# Autodesk Inventor assembly: leg_1
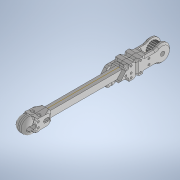
[picture p0: Inventor's stored thumbnail of the model, 180x180]
Saved by Autodesk Inventor 2020 (Build 240168000, 168)
## iProperties
Created: 2019-05-01
Part Number: leg_1
Document SubType Name: Assembly
Designer: psrob
Author: psrob
## Documents named in this file (8)
- E:\projects-2\project dog gen2\hardware\leg_bone_1.iam
- E:\projects-2\project dog gen2\hardware\leg_down_2.ipt
- E:\projects-2\project dog gen2\hardware\carbon_fiber_6.ipt
- E:\projects-2\project dog gen2\hardware\leg_down_3.ipt
- E:\projects-2\project dog gen2\hardware\leg_hip_1.ipt
- E:\projects-2\project dog gen2\hardware\leg_down_s1.ipt
- E:\projects-2\project dog gen2\hardware\leg_down_s1_MIR.ipt
- E:\projects-2\project dog gen2\hardware\leg_down_s3_l.ipt
## Components (8 placed, 7 different names)
1. carbon_fiber_6:1 — Mate:1, Mate:2, Mate:3, Flush:1, Mate:4, Mate:5, Flush:2, Mate:6, Mate:8, Mate:9
2. leg_down_2:1 — Mate:1, Mate:2, Mate:3, Insert:1, Insert:2, Mate:10
3. leg_down_3:1 — Insert:1, Insert:2, Mate:7
4. leg_hip_1:1 — Flush:1, Mate:4, Mate:5, Insert:3, Insert:4
5. leg_hip_1:2 — Insert:3, Insert:4
6. leg_down_s1:1 — Flush:2, Mate:6, Mate:7, Mate:11, Insert:5, Insert:6
7. leg_down_s1_MIR:1 — Mate:8, Mate:9, Mate:10
8. leg_down_s3_l:1 — Mate:11, Insert:5, Insert:6
## Relationships (19: Mate 11, Insert 6, Flush 2)
- Mate:1: carbon_fiber_6:1 ↔ leg_down_2:1
- Mate:2: carbon_fiber_6:1 ↔ leg_down_2:1
- Mate:3: carbon_fiber_6:1 ↔ leg_down_2:1
- Insert:1: leg_down_2:1 ↔ leg_down_3:1
- Insert:2: leg_down_2:1 ↔ leg_down_3:1
- Flush:1: carbon_fiber_6:1 ↔ leg_hip_1:1
- Mate:4: carbon_fiber_6:1 ↔ leg_hip_1:1
- Mate:5: carbon_fiber_6:1 ↔ leg_hip_1:1
- Insert:3: leg_hip_1:1 ↔ leg_hip_1:2
- Insert:4: leg_hip_1:1 ↔ leg_hip_1:2
- Flush:2: carbon_fiber_6:1 ↔ leg_down_s1:1
- Mate:6: carbon_fiber_6:1 ↔ leg_down_s1:1
- Mate:7: leg_down_3:1 ↔ leg_down_s1:1
- Mate:8: carbon_fiber_6:1 ↔ leg_down_s1_MIR:1
- Mate:9: carbon_fiber_6:1 ↔ leg_down_s1_MIR:1
- Mate:10: leg_down_2:1 ↔ leg_down_s1_MIR:1
- Mate:11: leg_down_s1:1 ↔ leg_down_s3_l:1
- Insert:5: leg_down_s1:1 ↔ leg_down_s3_l:1
- Insert:6: leg_down_s1:1 ↔ leg_down_s3_l:1
